# Autodesk Inventor assembly: SpurLarge
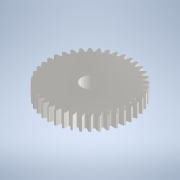
[picture p0: Inventor's stored thumbnail of the model, 180x180]
Saved by Autodesk Inventor 2022 (Build 260153000, 153)
## iProperties
Created: 2023-02-07
Part Number: SpurLarge
Document SubType Name: Assembly
Designer: Deven Joshi
Author: Deven Joshi
## Documents named in this file (2)
- C:\Users\ac_jo\OneDrive\Documents\TA202\SpurLarge.iam
- C:\Users\ac_jo\OneDrive\Documents\TA202\SpurLarge\Design Accelerator\Spur Gears2.iam
## Components (1 placed, 1 different names)
1. Spur Gears:2 [sub-assembly] — Mate:1
## Relationships (1: Mate 1)
- Mate:1: Spur Gears:2
